# Autodesk Inventor assembly: NDV-2000 Collector 01
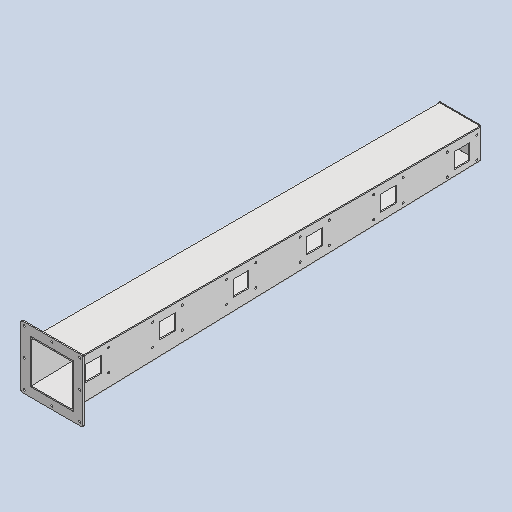
[picture p0: Inventor's stored thumbnail of the model, 512x512]
Saved by Autodesk Inventor 2026.2 (Build 302298000, 298)
## iProperties
Created: 2026-05-12
Part Number: NDV-2000 Collector 01
Document SubType Name: Assembly
Designer: admin
Stock Number: Коллектор
Author: admin
## Documents named in this file (5)
- C:\Users\admin\Documents\Inventor\NDV-DistribSystem\DRS_D1200\NDV-2000 Collector 01.iam
- C:\Users\admin\Documents\Inventor\NDV-DistribSystem\DRS_D1200\NDV-2102 Collector top 01.ipt
- C:\Users\admin\Documents\Inventor\NDV-DistribSystem\DRS_D1200\NDV-2101 Collector bottom 01.ipt
- C:\Users\admin\Documents\Inventor\NDV-DistribSystem\DRS_D1200\NDV-2104 Collector cap 01.ipt
- C:\Users\admin\Documents\Inventor\NDV-DistribSystem\DRS_D1200\NDV-2103 Collector flange 01.ipt
## Components (4 placed, 4 different names)
1. NDV-2102 Collector top 01:1 — Flush:10, Flush:9, Mate:11, Rigid:23, Mate:108
2. NDV-2101 Collector bottom 01:1 — Rigid:23, Mate:107, Flush:43
3. NDV-2104 Collector cap 01:1 — Flush:10, Flush:9, Mate:11
4. NDV-2103 Collector flange 01:1 — Mate:107, Mate:108, Flush:43
## Relationships (7: Flush 3, Mate 3, WeldJoint 1)
- Flush:10 (1 mm): NDV-2102 Collector top 01:1 ↔ NDV-2104 Collector cap 01:1
- Flush:9 (-1 mm): NDV-2102 Collector top 01:1 ↔ NDV-2104 Collector cap 01:1
- Mate:11: NDV-2102 Collector top 01:1 ↔ NDV-2104 Collector cap 01:1
- Rigid:23 [WeldJoint]: NDV-2102 Collector top 01:1 ↔ NDV-2101 Collector bottom 01:1
- Mate:107 (0.1 mm): NDV-2101 Collector bottom 01:1 ↔ NDV-2103 Collector flange 01:1
- Mate:108 (0.1 mm): NDV-2102 Collector top 01:1 ↔ NDV-2103 Collector flange 01:1
- Flush:43: NDV-2101 Collector bottom 01:1 ↔ NDV-2103 Collector flange 01:1
